# Autodesk Inventor assembly: Overall_Assembly_Rev3
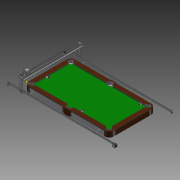
[picture p0: Inventor's stored thumbnail of the model, 180x180]
Saved by Autodesk Inventor 2015 (Build 190159000, 159)
## iProperties
Created: 2017-01-22
Part Number: Overall_Assembly_Rev3
Document SubType Name: Assembly
Designer: Guy
Author: Guy
## Documents named in this file (8)
- C:\Users\Guy\Documents\Fourth Year\Capstone\git\Capstone-Project\doc\CAD\LowLevel_Rev3\Overall_Assembly_Rev3.iam
- C:\Users\Guy\Documents\Fourth Year\Capstone\git\Capstone-Project\doc\CAD\Pool Table\Table_Model.ipt
- C:\Users\Guy\Documents\Fourth Year\Capstone\git\Capstone-Project\doc\CAD\LowLevel_Rev3\X_rail_Assembly_Rev3.iam
- C:\Users\Guy\Documents\Fourth Year\Capstone\git\Capstone-Project\doc\CAD\LowLevel_Rev3\Y_rail_Assembly_Rev3.iam
- C:\Users\Guy\Documents\Fourth Year\Capstone\git\Capstone-Project\doc\CAD\LowLevel_Rev3\Piston_Model.ipt
- C:\Users\Guy\Documents\Fourth Year\Capstone\git\Capstone-Project\doc\CAD\LowLevel_Rev2\Pool_Ball_Stripe.ipt
- C:\Users\Guy\Documents\Fourth Year\Capstone\git\Capstone-Project\doc\CAD\Nuts and Bolts\1-2in_13tpi x 8 in.ipt
- C:\Users\Guy\Documents\Fourth Year\Capstone\git\Capstone-Project\doc\CAD\Stepper Motor\NEMA 17\M1173041- NEMA 17.ipt
## Components (13 placed, 7 different names)
1. Table_Model:1 — Mate:2, Mate:4, Mate:5, Mate:7, Mate:8, Mate:9, Mate:15, Mate:16, Tangent:1, Tangent:2, Tangent:3, Tangent:4, Tangent:5, Tangent:6, Mate:33, Mate:35
2. X_rail_Assembly_Rev3:1 [sub-assembly] — Mate:2, Mate:4, Mate:5, Mate:7, Flush:1, Mate:16, Mate:30, Mate:32, Mate:34
3. X_rail_Assembly_Rev3:2 [sub-assembly] — Mate:8, Mate:9, Flush:1, Mate:15, Mate:27, Mate:31, Mate:36, Mate:37, Mate:38, Mate:39
4. Y_rail_Assembly_Rev3:1 [sub-assembly] — Mate:27, Mate:29, Flush:2, Mate:30, Mate:31, Mate:40, Flush:3
5. Pool_Ball_Stripe:1 — Tangent:1, Tangent:2
6. Pool_Ball_Stripe:2 — Tangent:3, Tangent:4
7. Pool_Ball_Stripe:3 — Tangent:5, Tangent:6
8. Piston_Model:1 — Mate:29, Flush:2
9. 1-2in_13tpi x 8 in:1 — Mate:32, Mate:33
10. 1-2in_13tpi x 8 in:2 — Mate:34, Mate:35
11. 1-2in_13tpi x 8 in:3 — Mate:36, Mate:37
12. 1-2in_13tpi x 8 in:4 — Mate:38, Mate:39
13. M1173041- NEMA 17:1 — Mate:40, Flush:3
## Relationships (30: Mate 21, Tangent 6, Flush 3)
- Mate:2: Table_Model:1 ↔ X_rail_Assembly_Rev3:1
- Mate:4: Table_Model:1 ↔ X_rail_Assembly_Rev3:1
- Mate:5: Table_Model:1 ↔ X_rail_Assembly_Rev3:1
- Mate:7: Table_Model:1 ↔ X_rail_Assembly_Rev3:1
- Mate:8: Table_Model:1 ↔ X_rail_Assembly_Rev3:2
- Mate:9: Table_Model:1 ↔ X_rail_Assembly_Rev3:2
- Flush:1: X_rail_Assembly_Rev3:1 ↔ X_rail_Assembly_Rev3:2
- Mate:15 (130 mm): Table_Model:1 ↔ X_rail_Assembly_Rev3:2
- Mate:16 (130 mm): Table_Model:1 ↔ X_rail_Assembly_Rev3:1
- Tangent:1: Table_Model:1 ↔ Pool_Ball_Stripe:1
- Tangent:2: Table_Model:1 ↔ Pool_Ball_Stripe:1
- Tangent:3: Table_Model:1 ↔ Pool_Ball_Stripe:2
- Tangent:4: Table_Model:1 ↔ Pool_Ball_Stripe:2
- Tangent:5: Table_Model:1 ↔ Pool_Ball_Stripe:3
- Tangent:6: Table_Model:1 ↔ Pool_Ball_Stripe:3
- Mate:27: X_rail_Assembly_Rev3:2 ↔ Y_rail_Assembly_Rev3:1
- Mate:29: Y_rail_Assembly_Rev3:1 ↔ Piston_Model:1
- Flush:2: Y_rail_Assembly_Rev3:1 ↔ Piston_Model:1
- Mate:30: X_rail_Assembly_Rev3:1 ↔ Y_rail_Assembly_Rev3:1
- Mate:31: X_rail_Assembly_Rev3:2 ↔ Y_rail_Assembly_Rev3:1
- Mate:32: X_rail_Assembly_Rev3:1 ↔ 1-2in_13tpi x 8 in:1
- Mate:33: Table_Model:1 ↔ 1-2in_13tpi x 8 in:1
- Mate:34: X_rail_Assembly_Rev3:1 ↔ 1-2in_13tpi x 8 in:2
- Mate:35: Table_Model:1 ↔ 1-2in_13tpi x 8 in:2
- Mate:36: X_rail_Assembly_Rev3:2 ↔ 1-2in_13tpi x 8 in:3
- Mate:37: X_rail_Assembly_Rev3:2 ↔ 1-2in_13tpi x 8 in:3
- Mate:38: X_rail_Assembly_Rev3:2 ↔ 1-2in_13tpi x 8 in:4
- Mate:39: X_rail_Assembly_Rev3:2 ↔ 1-2in_13tpi x 8 in:4
- Mate:40: Y_rail_Assembly_Rev3:1 ↔ M1173041- NEMA 17:1
- Flush:3: Y_rail_Assembly_Rev3:1 ↔ M1173041- NEMA 17:1
